# Autodesk Inventor assembly: y_carriage
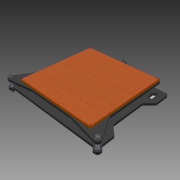
[picture p0: Inventor's stored thumbnail of the model, 180x180]
Saved by Autodesk Inventor 2014 (Build 180170000, 170)
## iProperties
Created: 2014-03-29
Part Number: y_carriage
Document SubType Name: Assembly
Designer: buben
Author: buben
## Documents named in this file (11)
- C:\Users\buben\Documents\GitHub\bacon\inventor files\printer parts\6.5 mm\y_carriage.iam
- C:\Users\buben\Documents\GitHub\bacon\inventor files\printer parts\6.5 mm\y_carriage.ipt
- C:\Users\buben\Documents\GitHub\bacon\inventor files\printer parts\6.5 mm\heatbed_mount.ipt
- C:\Users\buben\Documents\GitHub\bacon\inventor files\utils\washer_m5.ipt
- C:\Users\buben\Documents\Inventor\Content Center Files\R2014\en-US\ISO 4762(2)\ISO 4762 - M5 x 40ISO.ipt
- C:\Users\buben\Documents\GitHub\bacon\inventor files\assemblies\y_carryage\Design Accelerator\Compress Spring1.iam
- C:\Users\buben\Documents\GitHub\bacon\inventor files\utils\heatbed_thermal_insulation.ipt
- C:\Users\buben\Documents\GitHub\bacon\inventor files\utils\pcb_heatbed.ipt
- C:\Users\buben\Documents\GitHub\bacon\inventor files\3rd party components\linear_bearing_8\Imported Components\LU8MM\LU8MM.iam
- C:\Users\buben\Documents\GitHub\bacon\inventor files\printer parts\6.5 mm\y_carriage_belt_mount.ipt
- C:\Users\buben\Documents\GitHub\bacon\inventor files\printer parts\6.5 mm\y_carriage_belt_mount_bed_holder.ipt
## Components (29 placed, 10 different names)
1. y_carriage:1 — Mate:1, Mate:2, Mate:9, Mate:10, Mate:11, Mate:15, Mate:16, Mate:17, Mate:40, Flush:1, Flush:2, Mate:41, Mate:42, Mate:43, Mate:44, Mate:47, Mate:48, Mate:49, Mate:50, Mate:57, Mate:58, Mate:59
2. heatbed_mount:1 — Mate:1, Mate:2, Mate:3, Mate:4, Mate:5, Mate:6, Mate:7, Mate:8, Mate:12, Mate:13, Mate:14, Mate:34, Mate:35, Mate:36
3. CSN 02 1702 B B 5,3:1 — Mate:5, Mate:6, Insert:3
4. CSN 02 1702 B B 5,3:2 — Mate:4, Mate:7, Insert:2
5. CSN 02 1702 B B 5,3:3 — Mate:3, Mate:8, Insert:1
6. CSN 02 1702 B B 5,3:4 — Mate:9, Mate:24, Mate:29, Mate:30
7. CSN 02 1702 B B 5,3:5 — Mate:10, Mate:25, Mate:27, Mate:32
8. CSN 02 1702 B B 5,3:6 — Mate:13, Mate:18, Mate:33
9. CSN 02 1702 B B 5,3:7 — Mate:14, Mate:20
10. CSN 02 1702 B B 5,3:8 — Mate:11, Mate:26, Mate:28, Mate:31
11. CSN 02 1702 B B 5,3:9 — Mate:15, Mate:21
12. CSN 02 1702 B B 5,3:10 — Mate:17, Mate:22
13. CSN 02 1702 B B 5,3:11 — Mate:16, Mate:23
14. CSN 02 1702 B B 5,3:12 — Mate:12, Mate:19
15. ISO 4762 M5 x 40:1 — Insert:1, Mate:19, Mate:23, Mate:24
16. ISO 4762 M5 x 40:2 — Insert:2, Mate:18, Mate:22, Mate:25
17. ISO 4762 M5 x 40:3 — Insert:3, Mate:20, Mate:21, Mate:26
18. Compress Spring:1 [sub-assembly] — Mate:27, Mate:32, Mate:33
19. Compress Spring:2 [sub-assembly] — Mate:29, Mate:30
20. Compress Spring:3 [sub-assembly] — Mate:28, Mate:31
21. heatbed_thermal_insulation:1 — Mate:34, Mate:35, Mate:36, Mate:37, Mate:38, Mate:39
22. pcb_heatbed:1 — Mate:37, Mate:38, Mate:39
23. LU8MM:1 [sub-assembly] — Mate:41, Mate:42, Mate:46, Mate:48
24. LU8MM:2 [sub-assembly] — Mate:43, Mate:44, Mate:45, Mate:47
25. LU8MM:3 [sub-assembly] — Mate:45, Mate:50
26. LU8MM:4 [sub-assembly] — Mate:46, Mate:49
27. y_carriage_belt_mount:1 — Mate:52, Mate:54, Mate:56, Mate:57, Mate:58
28. y_carriage_belt_mount:2 — Mate:51, Mate:53, Mate:55, Mate:59
29. y_carriage_belt_mount_bed_holder:1 — Mate:51, Mate:52, Mate:53, Mate:54, Mate:55, Mate:56
## Relationships (64: Mate 59, Insert 3, Flush 2)
- Mate:1: y_carriage:1 ↔ heatbed_mount:1
- Mate:2: y_carriage:1 ↔ heatbed_mount:1
- Mate:3: heatbed_mount:1 ↔ CSN 02 1702 B B 5,3:3
- Mate:4: heatbed_mount:1 ↔ CSN 02 1702 B B 5,3:2
- Mate:5: heatbed_mount:1 ↔ CSN 02 1702 B B 5,3:1
- Mate:6: heatbed_mount:1 ↔ CSN 02 1702 B B 5,3:1
- Mate:7: heatbed_mount:1 ↔ CSN 02 1702 B B 5,3:2
- Mate:8: heatbed_mount:1 ↔ CSN 02 1702 B B 5,3:3
- Mate:9: y_carriage:1 ↔ CSN 02 1702 B B 5,3:4
- Mate:10: y_carriage:1 ↔ CSN 02 1702 B B 5,3:5
- Mate:11: y_carriage:1 ↔ CSN 02 1702 B B 5,3:8
- Mate:12: heatbed_mount:1 ↔ CSN 02 1702 B B 5,3:12
- Mate:13: heatbed_mount:1 ↔ CSN 02 1702 B B 5,3:6
- Mate:14: heatbed_mount:1 ↔ CSN 02 1702 B B 5,3:7
- Mate:15: y_carriage:1 ↔ CSN 02 1702 B B 5,3:9
- Mate:16: y_carriage:1 ↔ CSN 02 1702 B B 5,3:11
- Mate:17: y_carriage:1 ↔ CSN 02 1702 B B 5,3:10
- Insert:1: CSN 02 1702 B B 5,3:3 ↔ ISO 4762 M5 x 40:1
- Insert:2: CSN 02 1702 B B 5,3:2 ↔ ISO 4762 M5 x 40:2
- Insert:3: CSN 02 1702 B B 5,3:1 ↔ ISO 4762 M5 x 40:3
- Mate:18: CSN 02 1702 B B 5,3:6 ↔ ISO 4762 M5 x 40:2
- Mate:19: CSN 02 1702 B B 5,3:12 ↔ ISO 4762 M5 x 40:1
- Mate:20: CSN 02 1702 B B 5,3:7 ↔ ISO 4762 M5 x 40:3
- Mate:21: CSN 02 1702 B B 5,3:9 ↔ ISO 4762 M5 x 40:3
- Mate:22: CSN 02 1702 B B 5,3:10 ↔ ISO 4762 M5 x 40:2
- Mate:23: CSN 02 1702 B B 5,3:11 ↔ ISO 4762 M5 x 40:1
- Mate:24: CSN 02 1702 B B 5,3:4 ↔ ISO 4762 M5 x 40:1
- Mate:25: CSN 02 1702 B B 5,3:5 ↔ ISO 4762 M5 x 40:2
- Mate:26: CSN 02 1702 B B 5,3:8 ↔ ISO 4762 M5 x 40:3
- Mate:27: CSN 02 1702 B B 5,3:5 ↔ Compress Spring:1
- Mate:28: CSN 02 1702 B B 5,3:8 ↔ Compress Spring:3
- Mate:29: CSN 02 1702 B B 5,3:4 ↔ Compress Spring:2
- Mate:30: CSN 02 1702 B B 5,3:4 ↔ Compress Spring:2
- Mate:31: CSN 02 1702 B B 5,3:8 ↔ Compress Spring:3
- Mate:32: CSN 02 1702 B B 5,3:5 ↔ Compress Spring:1
- Mate:33: CSN 02 1702 B B 5,3:6 ↔ Compress Spring:1
- Mate:34: heatbed_mount:1 ↔ heatbed_thermal_insulation:1
- Mate:35: heatbed_mount:1 ↔ heatbed_thermal_insulation:1
- Mate:36: heatbed_mount:1 ↔ heatbed_thermal_insulation:1
- Mate:37: heatbed_thermal_insulation:1 ↔ pcb_heatbed:1
- Mate:38: heatbed_thermal_insulation:1 ↔ pcb_heatbed:1
- Mate:39: heatbed_thermal_insulation:1 ↔ pcb_heatbed:1
- Mate:40: y_carriage:1
- Flush:1: y_carriage:1
- Flush:2: y_carriage:1
- Mate:41 (7.5 mm): y_carriage:1 ↔ LU8MM:1
- Mate:42 (7.5 mm): y_carriage:1 ↔ LU8MM:1
- Mate:43 (7.5 mm): y_carriage:1 ↔ LU8MM:2
- Mate:44 (7.5 mm): y_carriage:1 ↔ LU8MM:2
- Mate:45: LU8MM:2 ↔ LU8MM:3
- Mate:46: LU8MM:1 ↔ LU8MM:4
- Mate:47 (0.5 mm): y_carriage:1 ↔ LU8MM:2
- Mate:48 (0.5 mm): y_carriage:1 ↔ LU8MM:1
- Mate:49 (0.5 mm): y_carriage:1 ↔ LU8MM:4
- Mate:50 (0.5 mm): y_carriage:1 ↔ LU8MM:3
- Mate:51: y_carriage_belt_mount:2 ↔ y_carriage_belt_mount_bed_holder:1
- Mate:52: y_carriage_belt_mount:1 ↔ y_carriage_belt_mount_bed_holder:1
- Mate:53: y_carriage_belt_mount:2 ↔ y_carriage_belt_mount_bed_holder:1
- Mate:54: y_carriage_belt_mount:1 ↔ y_carriage_belt_mount_bed_holder:1
- Mate:55: y_carriage_belt_mount:2 ↔ y_carriage_belt_mount_bed_holder:1
- Mate:56: y_carriage_belt_mount:1 ↔ y_carriage_belt_mount_bed_holder:1
- Mate:57: y_carriage:1 ↔ y_carriage_belt_mount:1
- Mate:58: y_carriage:1 ↔ y_carriage_belt_mount:1
- Mate:59: y_carriage:1 ↔ y_carriage_belt_mount:2
